# Autodesk Inventor assembly: Assembly_spindeldrive_350mm
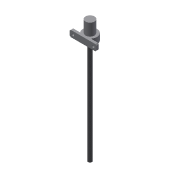
[picture p0: Inventor's stored thumbnail of the model, 180x180]
Saved by Autodesk Inventor 2019.4 (Build 234330000, 330)
## iProperties
Created: 2020-10-27
Part Number: Assembly_spindeldrive_350mm
Document SubType Name: Assembly
Designer: diederichbenedict
Author: diederichbenedict
## Documents named in this file (3)
- C:\Users\diederichbenedict\Dropbox\Dokumente\Promotion\PROJECTS\OPENTRONS\INVENTOR\Assembly_spindeldrive_350mm.iam
- C:\Users\diederichbenedict\Dropbox\Dokumente\Promotion\PROJECTS\OPENTRONS\INVENTOR\00_spindel_350mm.ipt
- C:\Users\diederichbenedict\Dropbox\Dokumente\Promotion\PROJECTS\OPENTRONS\INVENTOR\00_spindel_bearings.ipt
## Components (2 placed, 2 different names)
1. 00_spindel_350mm:1 — Mate:1, Mate:6
2. 00_spindel_bearings:2 — Mate:1, Angle:1, Mate:6
## Relationships (3: Mate 2, Angle 1)
- Mate:1: 00_spindel_350mm:1 ↔ 00_spindel_bearings:2
- Angle:1 (180 deg): 00_spindel_bearings:2
- Mate:6: 00_spindel_350mm:1 ↔ 00_spindel_bearings:2
